# Autodesk Inventor assembly: 800-MOTOR-CONTROLLER-PACK
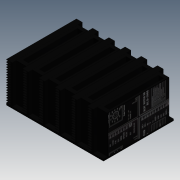
[picture p0: Inventor's stored thumbnail of the model, 180x180]
Saved by Autodesk Inventor 2018.2 (Build 222227000, 227)
## iProperties
Manager: feesmrt
Company: FRANCOR
Part Number: 800-MOTOR-CONTROLLER-PACK
Project: Rescue Robot
Cost Center: -
Material: Generisch
Document SubType Name: Assembly
Designer: feesmrt
Engineer: feesmrt
Authority: feesmrt
Subject: Rescue Robot
Author: feesmrt
Revision Number: 1
## Documents named in this file (2)
- D:\Programmierung\FRANC0R\CAD\02-Rocker-Bogie-Robot\800-ELECTRONICS\800-MOTOR-CONTROLLER-PACK.iam
- D:\Programmierung\FRANC0R\CAD\02-Rocker-Bogie-Robot\800-ELECTRONICS\800-20-MOTOR-CONTROLLER\800-20-MOTOR-CONTROLLER-BLD-300B.iam
## Components (6 placed, 1 different names)
1. 800-20-MOTOR-CONTROLLER-BLD-300B:1 [sub-assembly] — Passend:1, Passend:2
2. 800-20-MOTOR-CONTROLLER-BLD-300B:2 [sub-assembly]
3. 800-20-MOTOR-CONTROLLER-BLD-300B:3 [sub-assembly]
4. 800-20-MOTOR-CONTROLLER-BLD-300B:4 [sub-assembly]
5. 800-20-MOTOR-CONTROLLER-BLD-300B:5 [sub-assembly]
6. 800-20-MOTOR-CONTROLLER-BLD-300B:6 [sub-assembly]
## Component patterns: (6 elements, first: 800-20-MOTOR-CONTROLLER-BLD-300B:1)
## Relationships (2: Mate 2)
- Passend:1 [Mate]: 800-20-MOTOR-CONTROLLER-BLD-300B:1
- Passend:2 [Mate]: 800-20-MOTOR-CONTROLLER-BLD-300B:1
